# Autodesk Inventor assembly: 어셈블리
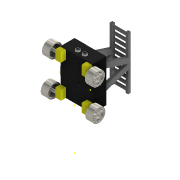
[picture p0: Inventor's stored thumbnail of the model, 180x180]
Saved by Autodesk Inventor 2020 (Build 240168000, 168)
## iProperties
Created: 2022-08-25
Part Number: 어셈블리
Document SubType Name: Assembly
Designer: 박연호
Author: 박연호
## Documents named in this file (10)
- C:\Users\박연호\OneDrive\바탕 화면\신산업\어셈블리.iam
- C:\Users\박연호\OneDrive\바탕 화면\신산업\레이저\본체 겉면 레이저 앞판.ipt
- C:\Users\박연호\OneDrive\바탕 화면\신산업\레이저\본체 겉면 레이저 옆판.ipt
- C:\Users\박연호\OneDrive\바탕 화면\신산업\레이저\본체 뚜껑 레이저.ipt
- C:\Users\박연호\OneDrive\바탕 화면\신산업\레이저\본체 밑판 레이저.ipt
- C:\Users\박연호\OneDrive\바탕 화면\신산업\빨랫대.ipt
- C:\Users\박연호\OneDrive\바탕 화면\신산업\레이저\모터.ipt
- C:\Users\박연호\OneDrive\바탕 화면\신산업\레이저\바퀴.ipt
- C:\Users\박연호\Downloads\hc-sr04.ipt
- C:\Users\박연호\Downloads\$_B_@578AB_@_5528.ipt
## Components (18 placed, 9 different names)
1. 본체 겉면 레이저 앞판:1 — 메이트:1, 메이트:2, 메이트:3, 메이트:8, 플러쉬:3, 플러쉬:4, 플러쉬:5, 플러쉬:7, 메이트:12, 플러쉬:11, 플러쉬:12, 메이트:23
2. 본체 겉면 레이저 앞판:2 — 메이트:5, 메이트:6, 메이트:9, 플러쉬:1, 플러쉬:2, 플러쉬:6, 플러쉬:8, 플러쉬:13, 플러쉬:15, 메이트:22
3. 본체 겉면 레이저 옆판:1 — 메이트:3, 메이트:4, 메이트:5, 플러쉬:2, 플러쉬:4, 메이트:10, 플러쉬:10, 플러쉬:14
4. 본체 겉면 레이저 옆판:2 — 메이트:7, 메이트:8, 메이트:9, 플러쉬:1, 플러쉬:3, 메이트:11, 플러쉬:9, 플러쉬:16
5. 본체 뚜껑 레이저:1 — 메이트:10, 메이트:11, 메이트:12, 메이트:13
6. 본체 밑판 레이저:1 — 메이트:1, 메이트:2, 메이트:4, 메이트:6, 메이트:7, 플러쉬:5, 플러쉬:6, 플러쉬:7, 플러쉬:8, 메이트:14, 메이트:15, 메이트:16, 메이트:17
7. 빨랫대:1 — 메이트:13, 메이트:24
8. 모터:1 — 메이트:17, 플러쉬:15, 플러쉬:16, 메이트:20
9. 모터:2 — 플러쉬:10, 메이트:15, 플러쉬:11, 메이트:18
10. 모터:3 — 메이트:16, 플러쉬:13, 플러쉬:14, 메이트:19
11. 모터:4 — 메이트:14, 플러쉬:9, 플러쉬:12, 메이트:21
12. 바퀴:1 — 메이트:18
13. 바퀴:2 — 메이트:19
14. 바퀴:3 — 메이트:21
15. 바퀴:4 — 메이트:20
16. hc-sr04:1 — 메이트:22
17. hc-sr04:2 — 메이트:23
18. $_B_@578AB_@_5528:1 — 메이트:24
## Relationships (40: Mate 24, Flush 16)
- 메이트:1 [Mate]: 본체 겉면 레이저 앞판:1 ↔ 본체 밑판 레이저:1
- 메이트:2 [Mate]: 본체 겉면 레이저 앞판:1 ↔ 본체 밑판 레이저:1
- 메이트:3 [Mate]: 본체 겉면 레이저 앞판:1 ↔ 본체 겉면 레이저 옆판:1
- 메이트:4 [Mate]: 본체 겉면 레이저 옆판:1 ↔ 본체 밑판 레이저:1
- 메이트:5 [Mate]: 본체 겉면 레이저 앞판:2 ↔ 본체 겉면 레이저 옆판:1
- 메이트:6 [Mate]: 본체 겉면 레이저 앞판:2 ↔ 본체 밑판 레이저:1
- 메이트:7 [Mate]: 본체 겉면 레이저 옆판:2 ↔ 본체 밑판 레이저:1
- 메이트:8 [Mate]: 본체 겉면 레이저 앞판:1 ↔ 본체 겉면 레이저 옆판:2
- 메이트:9 [Mate]: 본체 겉면 레이저 앞판:2 ↔ 본체 겉면 레이저 옆판:2
- 플러쉬:1 [Flush]: 본체 겉면 레이저 앞판:2 ↔ 본체 겉면 레이저 옆판:2
- 플러쉬:2 [Flush]: 본체 겉면 레이저 앞판:2 ↔ 본체 겉면 레이저 옆판:1
- 플러쉬:3 [Flush]: 본체 겉면 레이저 앞판:1 ↔ 본체 겉면 레이저 옆판:2
- 플러쉬:4 [Flush]: 본체 겉면 레이저 앞판:1 ↔ 본체 겉면 레이저 옆판:1
- 플러쉬:5 [Flush]: 본체 겉면 레이저 앞판:1 ↔ 본체 밑판 레이저:1
- 플러쉬:6 [Flush]: 본체 겉면 레이저 앞판:2 ↔ 본체 밑판 레이저:1
- 플러쉬:7 [Flush]: 본체 겉면 레이저 앞판:1 ↔ 본체 밑판 레이저:1
- 플러쉬:8 [Flush]: 본체 겉면 레이저 앞판:2 ↔ 본체 밑판 레이저:1
- 메이트:10 [Mate]: 본체 겉면 레이저 옆판:1 ↔ 본체 뚜껑 레이저:1
- 메이트:11 [Mate]: 본체 겉면 레이저 옆판:2 ↔ 본체 뚜껑 레이저:1
- 메이트:12 [Mate]: 본체 겉면 레이저 앞판:1 ↔ 본체 뚜껑 레이저:1
- 메이트:13 [Mate]: 본체 뚜껑 레이저:1 ↔ 빨랫대:1
- 메이트:14 [Mate]: 본체 밑판 레이저:1 ↔ 모터:4
- 플러쉬:9 [Flush]: 본체 겉면 레이저 옆판:2 ↔ 모터:4
- 플러쉬:10 [Flush]: 본체 겉면 레이저 옆판:1 ↔ 모터:2
- 메이트:15 [Mate]: 본체 밑판 레이저:1 ↔ 모터:2
- 플러쉬:11 [Flush]: 본체 겉면 레이저 앞판:1 ↔ 모터:2
- 플러쉬:12 [Flush]: 본체 겉면 레이저 앞판:1 ↔ 모터:4
- 메이트:16 [Mate]: 본체 밑판 레이저:1 ↔ 모터:3
- 플러쉬:13 [Flush]: 본체 겉면 레이저 앞판:2 ↔ 모터:3
- 플러쉬:14 [Flush]: 본체 겉면 레이저 옆판:1 ↔ 모터:3
- 메이트:17 [Mate]: 본체 밑판 레이저:1 ↔ 모터:1
- 플러쉬:15 [Flush]: 본체 겉면 레이저 앞판:2 ↔ 모터:1
- 플러쉬:16 [Flush]: 본체 겉면 레이저 옆판:2 ↔ 모터:1
- 메이트:18 [Mate]: 모터:2 ↔ 바퀴:1
- 메이트:19 [Mate]: 모터:3 ↔ 바퀴:2
- 메이트:20 [Mate]: 모터:1 ↔ 바퀴:4
- 메이트:21 [Mate]: 모터:4 ↔ 바퀴:3
- 메이트:22 [Mate] (5 mm): 본체 겉면 레이저 앞판:2 ↔ hc-sr04:1
- 메이트:23 [Mate] (5 mm): 본체 겉면 레이저 앞판:1 ↔ hc-sr04:2
- 메이트:24 [Mate]: 빨랫대:1 ↔ $_B_@578AB_@_5528:1
